# Autodesk Inventor assembly: completeRobot
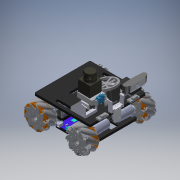
[picture p0: Inventor's stored thumbnail of the model, 180x180]
Saved by Autodesk Inventor 2017 (Build 210142000, 142)
## iProperties
Created: 2017-03-20
Part Number: completeRobot
Document SubType Name: Assembly
Designer: Naga
Author: Naga
## Documents named in this file (3)
- E:\GDrive\IEEE CS\SoutheastCon2017\Cad\completeRobot.iam
- E:\GDrive\IEEE CS\SoutheastCon2017\Cad\base.iam
- E:\GDrive\IEEE CS\SoutheastCon2017\Cad\top.iam
## Components (2 placed, 2 different names)
1. base:1 [sub-assembly] — Flush:1, Flush:2, Flush:3, Flush:4, Mate:1, Mate:2
2. top:1 [sub-assembly] — Flush:4, Mate:1, Mate:2
## Relationships (6: Flush 4, Mate 2)
- Flush:1: base:1
- Flush:2: base:1
- Flush:3: base:1
- Flush:4: base:1 ↔ top:1
- Mate:1: base:1 ↔ top:1
- Mate:2: base:1 ↔ top:1
